# Autodesk Inventor assembly: turret_assembly
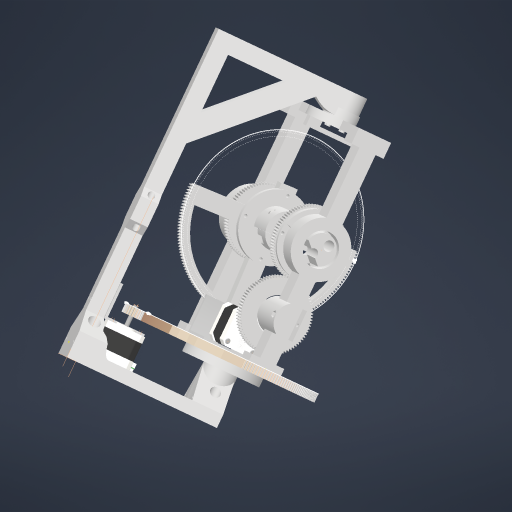
[picture p0: Inventor's stored thumbnail of the model, 512x512]
Saved by Autodesk Inventor 2023.2 (Build 272271000, 271)
## iProperties
Created: 2020-09-03
Part Number: turret_assembly
Document SubType Name: Assembly
Designer: bober
Author: bober
## Documents named in this file (20)
- F:\Turret\Our\Models\turret_assembly.iam
- F:\Turret\Our\Models\turret_assembly\Design Accelerator\vertical_axis_small_gear.ipt
- F:\Turret\Our\Models\turret_assembly\Design Accelerator\vertical_axis_bigl_gear.ipt
- F:\Turret\Our\Models\turret_assembly\Design Accelerator\horizontal_axis_big_gear.ipt
- F:\Turret\Our\Models\turret_assembly\Design Accelerator\pylon.ipt
- F:\Turret\Our\Models\turret_assembly\Design Accelerator\upper_grip.ipt
- F:\Turret\Our\Models\turret_assembly\Design Accelerator\main_stand_lower_half.ipt
- F:\Turret\Our\Models\turret_assembly\Design Accelerator\main_stand_upper_half.ipt
- F:\Turret\Our\Models\step_motor\Nema 17 Motor a Pasos 17HS4401.iam
- F:\Turret\Our\Models\turret_assembly\Design Accelerator\horizontal_lower_bearing_holder.ipt
- F:\Turret\Our\Models\turret_assembly\Design Accelerator\horizontal_axis_motor_metal_holder.ipt
- F:\Turret\Our\Models\turret_assembly\Design Accelerator\vertical_axis_motor_metal_holder.ipt
- F:\Turret\Our\Models\turret_assembly\Design Accelerator\Swash_distance.ipt
- F:\Turret\Our\Models\turret_assembly\Design Accelerator\big_actuator_holder.ipt
- F:\Turret\Our\Models\pylon_actuator_holder.ipt
- F:\Turret\Our\Models\pylon_actuator_holder_jaw.ipt
- F:\Turret\Our\Models\vertical_axis_hal_holder.ipt
- F:\Turret\Our\Models\turret_assembly\Design Accelerator\Spur Gears1.iam
- F:\Turret\Our\Models\turret_assembly\Design Accelerator\horizontal_axis_hal_gearr.ipt
- F:\Turret\Our\Models\pylon-hal-bearing-holder.ipt
## Components (25 placed, 19 different names)
1. vertical_axis_small_gear:1 — Tangent:1, Mate:4, Flush:1
2. horizontal_axis_big_gear:1 — Rigid:19, Insert:10
3. vertical_axis_small_gear:2 — Rotational:14
4. vertical_axis_bigl_gear:2 — Rigid:11, Rigid:12, Rigid:20, Tangent:1, Flush:1, Mate:6, Mate:7, Mate:9
5. pylon:2 — Rigid:20, Rigid:22, Insert:4
6. upper_grip:1 — Rigid:22, Flush:3, Insert:11, Insert:12
7. main_stand_lower_half:1 — Rigid:5, Rotational:12, Mate:1, Mate:2, Rigid:15, Mate:3
8. main_stand_upper_half:1 — Rigid:15
9. Nema 17 Motor a Pasos 17HS4401:2 [sub-assembly] — Mate:3, Mate:4
10. Nema 17 Motor a Pasos 17HS4401:3 [sub-assembly] — Rigid:13, Rotational:14
11. horizontal_lower_bearing_holder:1 — Rigid:11, Rotational:11
12. horizontal_axis_motor_metal_holder:1 — Rigid:12, Rigid:13
13. vertical_axis_motor_metal_holder:1 — Rigid:5
14. Swash_distance:1 — Rotational:11, Rotational:12
15. big_actuator_holder:1 — Rigid:19, Insert:2, Insert:3
16. pylon_actuator_holder:1 — Insert:6, Insert:2, Insert:3, Insert:7, Flush:4, Flush:5, Mate:5, Mate:8, Rotation:1
17. pylon_actuator_holder_jaw:1 — Insert:6, Insert:7
18. pylon_actuator_holder:2 — Insert:8, Insert:4, Insert:9, Insert:10
19. pylon_actuator_holder_jaw:2 — Insert:8, Insert:9
20. vertical_axis_hal_holder:1 — Flush:3, Insert:11, Insert:12
21. Spur Gears:1 [sub-assembly] — Flush:4
22. horizontal_axis_hal_gearr:1 — Flush:5, Mate:5, Mate:10, Mate:11, Mate:12, Mate:16, Rotation:1
23. pylon:3 — Mate:6, Mate:7, Mate:8, Mate:9, Flush:6, Mate:13, Mate:15
24. pylon-hal-bearing-holder:1 — Flush:6, Mate:13, Mate:15, Mate:16
25. vertical_axis_hal_holder:2 — Mate:10, Mate:11, Mate:12
## Relationships (43: Mate 15, Insert 10, WeldJoint 8, Flush 5, RevoluteJoint 3, Tangent 1, RelateRotation 1)
- Rigid:5 [WeldJoint]: main_stand_lower_half:1 ↔ vertical_axis_motor_metal_holder:1
- Rigid:11 [WeldJoint]: vertical_axis_bigl_gear:2 ↔ horizontal_lower_bearing_holder:1
- Rotational:11 [RevoluteJoint]: horizontal_lower_bearing_holder:1 ↔ Swash_distance:1
- Rotational:12 [RevoluteJoint]: main_stand_lower_half:1 ↔ Swash_distance:1
- Mate:1: main_stand_lower_half:1
- Mate:2: main_stand_lower_half:1
- Rigid:12 [WeldJoint]: vertical_axis_bigl_gear:2 ↔ horizontal_axis_motor_metal_holder:1
- Rigid:13 [WeldJoint]: Nema 17 Motor a Pasos 17HS4401:3 ↔ horizontal_axis_motor_metal_holder:1
- Rotational:14 [RevoluteJoint]: vertical_axis_small_gear:2 ↔ Nema 17 Motor a Pasos 17HS4401:3
- Rigid:15 [WeldJoint]: main_stand_lower_half:1 ↔ main_stand_upper_half:1
- Rigid:19 [WeldJoint]: horizontal_axis_big_gear:1 ↔ big_actuator_holder:1
- Rigid:20 [WeldJoint]: vertical_axis_bigl_gear:2 ↔ pylon:2
- Rigid:22 [WeldJoint]: pylon:2 ↔ upper_grip:1
- Tangent:1: vertical_axis_small_gear:1 ↔ vertical_axis_bigl_gear:2
- Mate:3: main_stand_lower_half:1 ↔ Nema 17 Motor a Pasos 17HS4401:2
- Mate:4: vertical_axis_small_gear:1 ↔ Nema 17 Motor a Pasos 17HS4401:2
- Flush:1: vertical_axis_small_gear:1 ↔ vertical_axis_bigl_gear:2
- Insert:6: pylon_actuator_holder:1 ↔ pylon_actuator_holder_jaw:1
- Insert:2 (-97.5 mm): big_actuator_holder:1 ↔ pylon_actuator_holder:1
- Insert:3 (-97.5 mm): big_actuator_holder:1 ↔ pylon_actuator_holder:1
- Insert:8: pylon_actuator_holder:2 ↔ pylon_actuator_holder_jaw:2
- Insert:4: pylon:2 ↔ pylon_actuator_holder:2
- Insert:7: pylon_actuator_holder:1 ↔ pylon_actuator_holder_jaw:1
- Insert:9: pylon_actuator_holder:2 ↔ pylon_actuator_holder_jaw:2
- Insert:10 (-30.5 mm): horizontal_axis_big_gear:1 ↔ pylon_actuator_holder:2
- Flush:3: upper_grip:1 ↔ vertical_axis_hal_holder:1
- Flush:4: pylon_actuator_holder:1 ↔ Spur Gears:1
- Insert:11: upper_grip:1 ↔ vertical_axis_hal_holder:1
- Insert:12: upper_grip:1 ↔ vertical_axis_hal_holder:1
- Flush:5: pylon_actuator_holder:1 ↔ horizontal_axis_hal_gearr:1
- Mate:5 (80 mm): pylon_actuator_holder:1 ↔ horizontal_axis_hal_gearr:1
- Mate:6: vertical_axis_bigl_gear:2 ↔ pylon:3
- Mate:7: vertical_axis_bigl_gear:2 ↔ pylon:3
- Mate:8: pylon_actuator_holder:1 ↔ pylon:3
- Mate:9: vertical_axis_bigl_gear:2 ↔ pylon:3
- Flush:6: pylon:3 ↔ pylon-hal-bearing-holder:1
- Mate:10: horizontal_axis_hal_gearr:1 ↔ vertical_axis_hal_holder:2
- Mate:11: horizontal_axis_hal_gearr:1 ↔ vertical_axis_hal_holder:2
- Mate:12: horizontal_axis_hal_gearr:1 ↔ vertical_axis_hal_holder:2
- Mate:13: pylon:3 ↔ pylon-hal-bearing-holder:1
- Mate:15 (0.07 mm): pylon:3 ↔ pylon-hal-bearing-holder:1
- Mate:16: horizontal_axis_hal_gearr:1 ↔ pylon-hal-bearing-holder:1
- Rotation:1 [RelateRotation] (1 ul): pylon_actuator_holder:1 ↔ horizontal_axis_hal_gearr:1
## Named parameters: d111_d107 = 0 mm
